# Autodesk Inventor assembly: 000-A-000
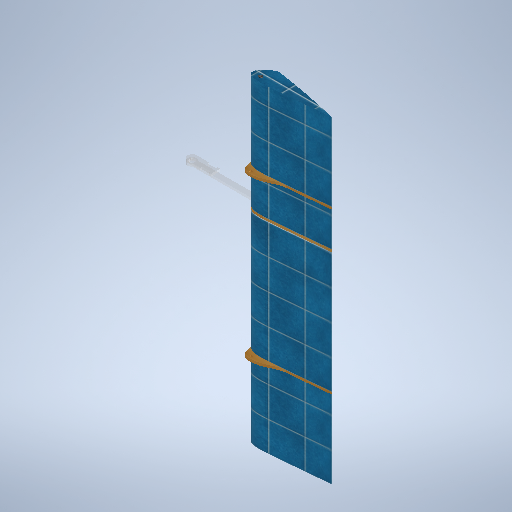
[picture p0: Inventor's stored thumbnail of the model, 512x512]
Saved by Autodesk Inventor 2025.2 (Build 292293000, 293)
## iProperties
Category: <PROJECT CATAGORY>
Created: 2025-01-30
Part Number: 000-A-000
Document SubType Name: Assembly
Designer: Carriett 4
Title: <TITLE>
Author: Carriett 4
Revision Number: A
## Documents named in this file (11)
- C:\Users\Carriett 4\OneDrive\CAD library\FLAP ASSEMBLY\FlapFinal v2\4A.01.01.04-BC-v1-Final Flap v2 Assembly.iam
- C:\Users\Carriett 4\OneDrive\CAD library\FLAP ASSEMBLY\FlapFinal v2\4P.01.01.14-BC-v1-Final Hinge Rib.ipt
- C:\Users\Carriett 4\OneDrive\CAD library\FLAP ASSEMBLY\FlapFinal v2\4P.01.01.15-BC-v1-Final Actuator Rib.ipt
- C:\Users\Carriett 4\OneDrive\CAD library\FLAP ASSEMBLY\FlapFinal v2\4P.01.01.16-BC-v1-Final Inboard Flap Foam.ipt
- C:\Users\Carriett 4\OneDrive\CAD library\FLAP ASSEMBLY\FlapFinal v2\4P.01.01.17-BC-v1-Final Middle Flap Foam.ipt
- C:\Users\Carriett 4\OneDrive\CAD library\FLAP ASSEMBLY\FlapFinal v2\4P.01.01.18-BC-v1-Final Middle2 Flap Foam.ipt
- C:\Users\Carriett 4\OneDrive\CAD library\FLAP ASSEMBLY\FlapFinal v2\4P.01.01.19-BC-v1-Final Outboard Flap Foam.ipt
- C:\Users\Carriett 4\OneDrive\CAD library\FLAP ASSEMBLY\FlapFinal v2\4P.01.01.20-BC-v1-Final Flap L2 80deg.ipt
- C:\Users\Carriett 4\OneDrive\CAD library\FLAP ASSEMBLY\FlapFinal v2\4P.01.01.21-BC-v1-Final Flap L3 80deg.ipt
- C:\Users\Carriett 4\OneDrive\CAD library\FLAP ASSEMBLY\FlapFinal v2\4P.01.01.15-BC-v1-Final Flap Spar.ipt
- C:\Users\me19654\OneDrive - University of Bristol\PhD Project\005 Design (CAD and schematics)\001 Wind Tunnel\CAD Library\001-A-017 CONTRACTION ASSY.iam
## Components (10 placed, 9 different names)
1. 4P.01.01.14-BC-v1-Final Hinge Rib:1 — Mate:5, Rigid:6, Mate:6, Rigid:7
2. 4P.01.01.14-BC-v1-Final Hinge Rib:2 — Mate:1, Rigid:2, Mate:2, Rigid:3
3. 4P.01.01.15-BC-v1-Final Actuator Rib:1 — Mate:3, Rigid:4, Mate:4, Rigid:5, Rotational:1
4. 4P.01.01.16-BC-v1-Final Inboard Flap Foam:1 — Rigid:1, Mate:1, Rigid:2
5. 4P.01.01.17-BC-v1-Final Middle Flap Foam:1 — Mate:2, Rigid:3, Mate:3, Rigid:4
6. 4P.01.01.18-BC-v1-Final Middle2 Flap Foam:1 — Mate:4, Rigid:5, Mate:5, Rigid:6
7. 4P.01.01.19-BC-v1-Final Outboard Flap Foam:1 — Mate:6, Rigid:7
8. 4P.01.01.20-BC-v1-Final Flap L2 80deg:1 — Rotational:2
9. 4P.01.01.21-BC-v1-Final Flap L3 80deg:1 — Rotational:1, Rotational:2
10. Flap Spar:1 — Rigid:1
## Relationships (15: WeldJoint 7, Mate 6, RevoluteJoint 2)
- Rigid:1 [WeldJoint]: 4P.01.01.16-BC-v1-Final Inboard Flap Foam:1 ↔ Flap Spar:1
- Mate:1: 4P.01.01.14-BC-v1-Final Hinge Rib:2 ↔ 4P.01.01.16-BC-v1-Final Inboard Flap Foam:1
- Rigid:2 [WeldJoint]: 4P.01.01.14-BC-v1-Final Hinge Rib:2 ↔ 4P.01.01.16-BC-v1-Final Inboard Flap Foam:1
- Mate:2: 4P.01.01.14-BC-v1-Final Hinge Rib:2 ↔ 4P.01.01.17-BC-v1-Final Middle Flap Foam:1
- Rigid:3 [WeldJoint]: 4P.01.01.14-BC-v1-Final Hinge Rib:2 ↔ 4P.01.01.17-BC-v1-Final Middle Flap Foam:1
- Mate:3: 4P.01.01.15-BC-v1-Final Actuator Rib:1 ↔ 4P.01.01.17-BC-v1-Final Middle Flap Foam:1
- Rigid:4 [WeldJoint]: 4P.01.01.15-BC-v1-Final Actuator Rib:1 ↔ 4P.01.01.17-BC-v1-Final Middle Flap Foam:1
- Mate:4: 4P.01.01.15-BC-v1-Final Actuator Rib:1 ↔ 4P.01.01.18-BC-v1-Final Middle2 Flap Foam:1
- Rigid:5 [WeldJoint]: 4P.01.01.15-BC-v1-Final Actuator Rib:1 ↔ 4P.01.01.18-BC-v1-Final Middle2 Flap Foam:1
- Mate:5: 4P.01.01.14-BC-v1-Final Hinge Rib:1 ↔ 4P.01.01.18-BC-v1-Final Middle2 Flap Foam:1
- Rigid:6 [WeldJoint]: 4P.01.01.14-BC-v1-Final Hinge Rib:1 ↔ 4P.01.01.18-BC-v1-Final Middle2 Flap Foam:1
- Mate:6: 4P.01.01.14-BC-v1-Final Hinge Rib:1 ↔ 4P.01.01.19-BC-v1-Final Outboard Flap Foam:1
- Rigid:7 [WeldJoint]: 4P.01.01.14-BC-v1-Final Hinge Rib:1 ↔ 4P.01.01.19-BC-v1-Final Outboard Flap Foam:1
- Rotational:1 [RevoluteJoint]: 4P.01.01.15-BC-v1-Final Actuator Rib:1 ↔ 4P.01.01.21-BC-v1-Final Flap L3 80deg:1
- Rotational:2 [RevoluteJoint]: 4P.01.01.20-BC-v1-Final Flap L2 80deg:1 ↔ 4P.01.01.21-BC-v1-Final Flap L3 80deg:1
